# Autodesk Inventor assembly: chain(b)
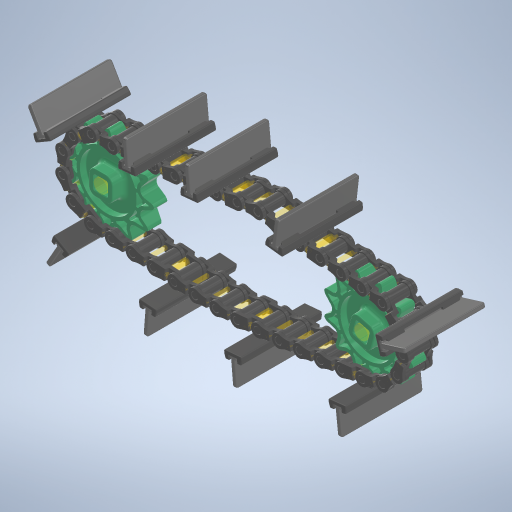
[picture p0: Inventor's stored thumbnail of the model, 512x512]
Saved by Autodesk Inventor 2023 (Build 270158000, 158)
## iProperties
Created: 2022-08-08
Part Number: chain(b)
Document SubType Name: Assembly
Designer: aaron
Author: aaron
## Documents named in this file (4)
- C:\Users\aaron\Documents\Inventor\Spin Up\library\Motion\New Sprockets\chain(b).iam
- C:\Users\aaron\Documents\Inventor\Spin Up\library\Motion\Sprockets\HS 12T Sprocket, No Insert.ipt
- C:\Users\aaron\Documents\Inventor\Spin Up\library\Motion\Chain + Tank Tread\High Strength Chain Link.ipt
- C:\Users\aaron\Documents\Inventor\Spin Up\library\Motion\Chain + Tank Tread\Short Flap.ipt
## Components (48 placed, 3 different names)
1. HS 12T Sprocket, No Insert:1 — Mate:1, Flush:1, Mate:34, Mate:35, Mate:36, Mate:37, Mate:38, Mate:39
2. HS 12T Sprocket, No Insert:2 — Mate:1, Flush:1, Mate:33, Flush:33, Mate:46, Mate:47, Mate:48, Mate:49, Mate:50
3. High Strength Chain Link:1 — Mate:2, Flush:2, Mate:33, Mate:51, Mate:58
4. High Strength Chain Link:2 — Mate:2, Flush:2, Mate:4, Flush:4, Flush:33, Flush:46
5. High Strength Chain Link:3 — Mate:4, Flush:4
6. High Strength Chain Link:4 — Mate:8, Flush:8
7. High Strength Chain Link:5 — Mate:8, Flush:8, Mate:57, Flush:45
8. High Strength Chain Link:6
9. High Strength Chain Link:7
10. High Strength Chain Link:8 — Mate:16, Flush:16
11. High Strength Chain Link:9 — Mate:16, Flush:16, Mate:56, Flush:44
12. High Strength Chain Link:10
13. High Strength Chain Link:11
14. High Strength Chain Link:12
15. High Strength Chain Link:13
16. High Strength Chain Link:14 — Mate:34, Mate:55
17. High Strength Chain Link:15 — Mate:35, Flush:41
18. High Strength Chain Link:16 — Mate:32, Flush:32, Mate:36
19. High Strength Chain Link:17 — Mate:32, Flush:32, Mate:37
20. High Strength Chain Link:18 — Mate:38, Mate:54
21. High Strength Chain Link:19 — Mate:39, Flush:42
22. High Strength Chain Link:20
23. High Strength Chain Link:21
24. High Strength Chain Link:22
25. High Strength Chain Link:23 — Mate:53
26. High Strength Chain Link:24 — Flush:43
27. High Strength Chain Link:25
28. High Strength Chain Link:26
29. High Strength Chain Link:27 — Mate:52, Flush:40
30. High Strength Chain Link:28
31. High Strength Chain Link:29
32. High Strength Chain Link:30 — Mate:60, Flush:48
33. High Strength Chain Link:31
34. High Strength Chain Link:32 — Mate:45, Flush:39, Mate:46
35. High Strength Chain Link:33 — Mate:45, Flush:39
36. High Strength Chain Link:34 — Mate:47, Mate:59
37. High Strength Chain Link:35 — Mate:48, Flush:47
38. High Strength Chain Link:36 — Mate:49
39. High Strength Chain Link:37 — Mate:50, Mate:51
40. Short Flap:1 — Mate:52, Flush:40
41. Short Flap:2 — Mate:53, Flush:43
42. Short Flap:3 — Mate:54, Flush:42
43. Short Flap:4 — Mate:55, Flush:41
44. Short Flap:5 — Mate:56, Flush:44
45. Short Flap:6 — Mate:57, Flush:45
46. Short Flap:7 — Mate:58, Flush:46
47. Short Flap:8 — Mate:59, Flush:47
48. Short Flap:9 — Mate:60, Flush:48
## Relationships (106: Mate 59, Flush 47)
- Mate:1 (121.92 mm): HS 12T Sprocket, No Insert:1 ↔ HS 12T Sprocket, No Insert:2
- Flush:1: HS 12T Sprocket, No Insert:1 ↔ HS 12T Sprocket, No Insert:2
- Mate:2: High Strength Chain Link:1 ↔ High Strength Chain Link:2
- Flush:2: High Strength Chain Link:1 ↔ High Strength Chain Link:2
- [Mate]: High Strength Chain Link:3 ↔ High Strength Chain Link:4
- [Flush]: High Strength Chain Link:3 ↔ High Strength Chain Link:4
- Mate:4: High Strength Chain Link:2 ↔ High Strength Chain Link:3
- Flush:4: High Strength Chain Link:2 ↔ High Strength Chain Link:3
- [Mate]: High Strength Chain Link:5 ↔ High Strength Chain Link:6
- [Flush]: High Strength Chain Link:5 ↔ High Strength Chain Link:6
- [Mate]: High Strength Chain Link:7 ↔ High Strength Chain Link:8
- [Flush]: High Strength Chain Link:7 ↔ High Strength Chain Link:8
- [Mate]: High Strength Chain Link:6 ↔ High Strength Chain Link:7
- [Flush]: High Strength Chain Link:6 ↔ High Strength Chain Link:7
- Mate:8: High Strength Chain Link:4 ↔ High Strength Chain Link:5
- Flush:8: High Strength Chain Link:4 ↔ High Strength Chain Link:5
- [Mate]: High Strength Chain Link:9 ↔ High Strength Chain Link:10
- [Flush]: High Strength Chain Link:9 ↔ High Strength Chain Link:10
- [Mate]: High Strength Chain Link:11 ↔ High Strength Chain Link:12
- [Flush]: High Strength Chain Link:11 ↔ High Strength Chain Link:12
- [Mate]: High Strength Chain Link:10 ↔ High Strength Chain Link:11
- [Flush]: High Strength Chain Link:10 ↔ High Strength Chain Link:11
- [Mate]: High Strength Chain Link:13 ↔ High Strength Chain Link:14
- [Flush]: High Strength Chain Link:13 ↔ High Strength Chain Link:14
- [Mate]: High Strength Chain Link:15 ↔ High Strength Chain Link:16
- [Flush]: High Strength Chain Link:15 ↔ High Strength Chain Link:16
- [Mate]: High Strength Chain Link:14 ↔ High Strength Chain Link:15
- [Flush]: High Strength Chain Link:14 ↔ High Strength Chain Link:15
- [Mate]: High Strength Chain Link:12 ↔ High Strength Chain Link:13
- [Flush]: High Strength Chain Link:12 ↔ High Strength Chain Link:13
- Mate:16: High Strength Chain Link:8 ↔ High Strength Chain Link:9
- Flush:16: High Strength Chain Link:8 ↔ High Strength Chain Link:9
- [Mate]: High Strength Chain Link:17 ↔ High Strength Chain Link:18
- [Flush]: High Strength Chain Link:17 ↔ High Strength Chain Link:18
- [Mate]: High Strength Chain Link:19 ↔ High Strength Chain Link:20
- [Flush]: High Strength Chain Link:19 ↔ High Strength Chain Link:20
- [Mate]: High Strength Chain Link:18 ↔ High Strength Chain Link:19
- [Flush]: High Strength Chain Link:18 ↔ High Strength Chain Link:19
- [Mate]: High Strength Chain Link:21 ↔ High Strength Chain Link:22
- [Flush]: High Strength Chain Link:21 ↔ High Strength Chain Link:22
- [Mate]: High Strength Chain Link:23 ↔ High Strength Chain Link:24
- [Flush]: High Strength Chain Link:23 ↔ High Strength Chain Link:24
- [Mate]: High Strength Chain Link:22 ↔ High Strength Chain Link:23
- [Flush]: High Strength Chain Link:22 ↔ High Strength Chain Link:23
- [Mate]: High Strength Chain Link:20 ↔ High Strength Chain Link:21
- [Flush]: High Strength Chain Link:20 ↔ High Strength Chain Link:21
- [Mate]: High Strength Chain Link:25 ↔ High Strength Chain Link:26
- [Flush]: High Strength Chain Link:25 ↔ High Strength Chain Link:26
- [Mate]: High Strength Chain Link:27 ↔ High Strength Chain Link:28
- [Flush]: High Strength Chain Link:27 ↔ High Strength Chain Link:28
- [Mate]: High Strength Chain Link:26 ↔ High Strength Chain Link:27
- [Flush]: High Strength Chain Link:26 ↔ High Strength Chain Link:27
- [Mate]: High Strength Chain Link:29 ↔ High Strength Chain Link:30
- [Flush]: High Strength Chain Link:29 ↔ High Strength Chain Link:30
- [Mate]: High Strength Chain Link:31 ↔ High Strength Chain Link:32
- [Flush]: High Strength Chain Link:31 ↔ High Strength Chain Link:32
- [Mate]: High Strength Chain Link:30 ↔ High Strength Chain Link:31
- [Flush]: High Strength Chain Link:30 ↔ High Strength Chain Link:31
- [Mate]: High Strength Chain Link:28 ↔ High Strength Chain Link:29
- [Flush]: High Strength Chain Link:28 ↔ High Strength Chain Link:29
- [Mate]: High Strength Chain Link:24 ↔ High Strength Chain Link:25
- [Flush]: High Strength Chain Link:24 ↔ High Strength Chain Link:25
- Mate:32: High Strength Chain Link:16 ↔ High Strength Chain Link:17
- Flush:32: High Strength Chain Link:16 ↔ High Strength Chain Link:17
- Mate:33: HS 12T Sprocket, No Insert:2 ↔ High Strength Chain Link:1
- Flush:33: HS 12T Sprocket, No Insert:2 ↔ High Strength Chain Link:2
- Mate:34: HS 12T Sprocket, No Insert:1 ↔ High Strength Chain Link:14
- Mate:35: HS 12T Sprocket, No Insert:1 ↔ High Strength Chain Link:15
- Mate:36: HS 12T Sprocket, No Insert:1 ↔ High Strength Chain Link:16
- Mate:37: HS 12T Sprocket, No Insert:1 ↔ High Strength Chain Link:17
- Mate:38: HS 12T Sprocket, No Insert:1 ↔ High Strength Chain Link:18
- Mate:39: HS 12T Sprocket, No Insert:1 ↔ High Strength Chain Link:19
- [Mate]: High Strength Chain Link:33 ↔ High Strength Chain Link:34
- [Flush]: High Strength Chain Link:33 ↔ High Strength Chain Link:34
- [Mate]: High Strength Chain Link:35 ↔ High Strength Chain Link:36
- [Flush]: High Strength Chain Link:35 ↔ High Strength Chain Link:36
- [Mate]: High Strength Chain Link:34 ↔ High Strength Chain Link:35
- [Flush]: High Strength Chain Link:34 ↔ High Strength Chain Link:35
- [Mate]: High Strength Chain Link:36 ↔ High Strength Chain Link:37
- [Flush]: High Strength Chain Link:36 ↔ High Strength Chain Link:37
- Mate:45: High Strength Chain Link:32 ↔ High Strength Chain Link:33
- Flush:39: High Strength Chain Link:32 ↔ High Strength Chain Link:33
- Mate:46: HS 12T Sprocket, No Insert:2 ↔ High Strength Chain Link:32
- Mate:47: HS 12T Sprocket, No Insert:2 ↔ High Strength Chain Link:34
- Mate:48: HS 12T Sprocket, No Insert:2 ↔ High Strength Chain Link:35
- Mate:49: HS 12T Sprocket, No Insert:2 ↔ High Strength Chain Link:36
- Mate:50: HS 12T Sprocket, No Insert:2 ↔ High Strength Chain Link:37
- Mate:51: High Strength Chain Link:1 ↔ High Strength Chain Link:37
- Mate:52: High Strength Chain Link:27 ↔ Short Flap:1
- Flush:40: High Strength Chain Link:27 ↔ Short Flap:1
- Mate:53: High Strength Chain Link:23 ↔ Short Flap:2
- Mate:54: High Strength Chain Link:18 ↔ Short Flap:3
- Mate:55: High Strength Chain Link:14 ↔ Short Flap:4
- Flush:41: High Strength Chain Link:15 ↔ Short Flap:4
- Flush:42: High Strength Chain Link:19 ↔ Short Flap:3
- Flush:43: High Strength Chain Link:24 ↔ Short Flap:2
- Mate:56: High Strength Chain Link:9 ↔ Short Flap:5
- Flush:44: High Strength Chain Link:9 ↔ Short Flap:5
- Mate:57: High Strength Chain Link:5 ↔ Short Flap:6
- Flush:45: High Strength Chain Link:5 ↔ Short Flap:6
- Mate:58: High Strength Chain Link:1 ↔ Short Flap:7
- Flush:46: High Strength Chain Link:2 ↔ Short Flap:7
- Mate:59: High Strength Chain Link:34 ↔ Short Flap:8
- Flush:47: High Strength Chain Link:35 ↔ Short Flap:8
- Mate:60: High Strength Chain Link:30 ↔ Short Flap:9
- Flush:48: High Strength Chain Link:30 ↔ Short Flap:9
## Named parameters: d4_d2 = 0 mm, d5_d3 = 0 mm, d8_d2 = 0 mm, d9_d3 = 0 mm, d10_d4_d2 = 0 mm, d11_d5_d3 = 0 mm, d12_d6 = 0 mm, d13_d7 = 0 mm, d16_d2 = 0 mm, d17_d3 = 0 mm, d18_d4_d2 = 0 mm, d19_d5_d3 = 0 mm, d20_d6 = 0 mm, d21_d7 = 0 mm, d22_d8_d2 = 0 mm, d23_d9_d3 = 0 mm, d24_d10_d4_d2 = 0 mm, d25_d11_d5_d3 = 0 mm, d26_d12_d6 = 0 mm, d27_d13_d7 = 0 mm, d28_d14 = 0 mm, d29_d15 = 0 mm, d32_d2 = 0 mm, d33_d3 = 0 mm, d34_d4_d2 = 0 mm, d35_d5_d3 = 0 mm, d36_d6 = 0 mm, d37_d7 = 0 mm, d38_d8_d2 = 0 mm, d39_d9_d3 = 0 mm, d40_d10_d4_d2 = 0 mm, d41_d11_d5_d3 = 0 mm, d42_d12_d6 = 0 mm, d43_d13_d7 = 0 mm, d44_d14 = 0 mm, d45_d15 = 0 mm, d46_d16_d2 = 0 mm, d47_d17_d3 = 0 mm, d48_d18_d4_d2 = 0 mm, d49_d19_d5_d3 = 0 mm, d50_d20_d6 = 0 mm, d51_d21_d7 = 0 mm, d52_d22_d8_d2 = 0 mm, d53_d23_d9_d3 = 0 mm, d54_d24_d10_d4_d2 = 0 mm, d55_d25_d11_d5_d3 = 0 mm, d56_d26_d12_d6 = 0 mm, d57_d27_d13_d7 = 0 mm, d58_d28_d14 = 0 mm, d59_d29_d15 = 0 mm, d60_d30 = 0 mm, d61_d31 = 0 mm, d72_d46_d16_d2 = 0 mm, d73_d47_d17_d3 = 0 mm, d74_d48_d18_d4_d2 = 0 mm, d75_d49_d19_d5_d3 = 0 mm, d76_d50_d20_d6 = 0 mm, d77_d51_d21_d7 = 0 mm, d80_d58_d28_d14 = 0 mm, d81_d59_d29_d15 = 0 mm
